# Autodesk Inventor assembly: 200-ROCKER-BOGIE-ASM
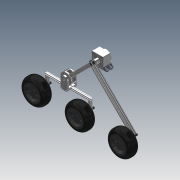
[picture p0: Inventor's stored thumbnail of the model, 180x180]
Saved by Autodesk Inventor 2018.2 (Build 222227000, 227)
## iProperties
Manager: feesmrt
Company: FRANC0R
Created: 2017-12-10
Part Number: 200-ROCKER-BOGIE-ASM
Material: Generisch
Document SubType Name: Assembly
Designer: feesmrt
Project: Rescue Robot
Description: Rocker Bogie Suspension
Engineer: feesmrt
Authority: feesmrt
Stock Number: 200-ROCKER-BOGIE-ASM
Author: feesmrt
Title: Rocker Bogie Suspension
Subject: Rescue Robot
Revision Number: 1
## Documents named in this file (4)
- D:\Programmierung\FRANC0R\CAD\02-Rocker-Bogie-Robot\200-ROCKER-BOGIE\200-ROCKER-BOGIE-ASM.iam
- D:\Programmierung\FRANC0R\CAD\02-Rocker-Bogie-Robot\200-ROCKER-BOGIE\200-ROCKER-ASM-01.iam
- D:\Programmierung\FRANC0R\CAD\02-Rocker-Bogie-Robot\200-ROCKER-BOGIE\200-BOGIE-ASM-01.iam
- D:\Programmierung\FRANC0R\CAD\02-Rocker-Bogie-Robot\900-COMPONENTS\900-10-WHEEL\900-10-WHEEL-ASM-01.iam
## Components (5 placed, 3 different names)
1. 200-ROCKER-ASM-01:1 [sub-assembly] — Passend:1, Passend:9, Passend:10, Passend:11, Passend:12, Passend:13, Passend:14, Passend:15
2. 200-BOGIE-ASM-01:1 [sub-assembly] — Passend:1, Passend:3, Passend:4, Passend:5, Passend:6, Passend:7, Passend:8, Passend:13, Passend:14, Passend:15
3. 900-10-WHEEL-ASM-01:1 [sub-assembly] — Passend:3, Passend:4, Passend:5
4. 900-10-WHEEL-ASM-01:2 [sub-assembly] — Passend:6, Passend:7, Passend:8
5. 900-10-WHEEL-ASM-01:3 [sub-assembly] — Passend:9, Passend:10, Passend:11, Passend:12
## Relationships (14: Mate 14)
- Passend:1 [Mate]: 200-ROCKER-ASM-01:1 ↔ 200-BOGIE-ASM-01:1
- Passend:3 [Mate]: 200-BOGIE-ASM-01:1 ↔ 900-10-WHEEL-ASM-01:1
- Passend:4 [Mate]: 200-BOGIE-ASM-01:1 ↔ 900-10-WHEEL-ASM-01:1
- Passend:5 [Mate]: 200-BOGIE-ASM-01:1 ↔ 900-10-WHEEL-ASM-01:1
- Passend:6 [Mate]: 200-BOGIE-ASM-01:1 ↔ 900-10-WHEEL-ASM-01:2
- Passend:7 [Mate]: 200-BOGIE-ASM-01:1 ↔ 900-10-WHEEL-ASM-01:2
- Passend:8 [Mate]: 200-BOGIE-ASM-01:1 ↔ 900-10-WHEEL-ASM-01:2
- Passend:9 [Mate]: 200-ROCKER-ASM-01:1 ↔ 900-10-WHEEL-ASM-01:3
- Passend:10 [Mate]: 200-ROCKER-ASM-01:1 ↔ 900-10-WHEEL-ASM-01:3
- Passend:11 [Mate]: 200-ROCKER-ASM-01:1 ↔ 900-10-WHEEL-ASM-01:3
- Passend:12 [Mate]: 200-ROCKER-ASM-01:1 ↔ 900-10-WHEEL-ASM-01:3
- Passend:13 [Mate]: 200-ROCKER-ASM-01:1 ↔ 200-BOGIE-ASM-01:1
- Passend:14 [Mate]: 200-ROCKER-ASM-01:1 ↔ 200-BOGIE-ASM-01:1
- Passend:15 [Mate]: 200-ROCKER-ASM-01:1 ↔ 200-BOGIE-ASM-01:1
